# Autodesk Inventor assembly: Batteriepack
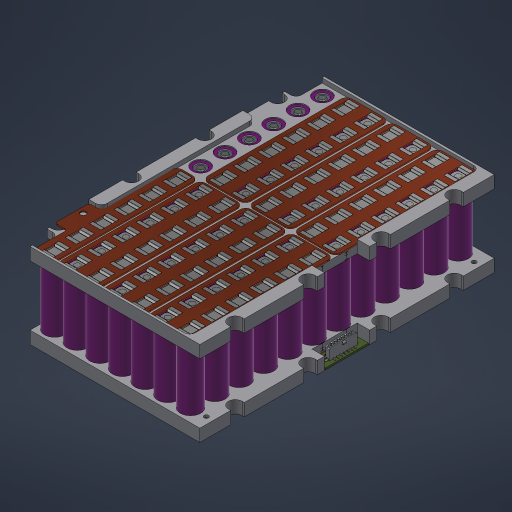
[picture p0: Inventor's stored thumbnail of the model, 512x512]
Saved by Autodesk Inventor 2024.3 (Build 283343010, 343A)
## iProperties
Created: 2025-03-26
Part Number: Batteriepack
Document SubType Name: Assembly
Designer: David Lill
Author: David Lill
## Documents named in this file (8)
- C:\Users\David\Documents\FTAG\E-16\Batterie\Batterie_Konstruktion\E-16 Batterie\Batteriepack.iam
- C:\Users\David\Documents\FTAG\E-16\Batterie\Batterie_Konstruktion\E-16 Batterie\Platte1.ipt
- C:\Users\David\Documents\FTAG\E-16\Batterie\Batterie_Konstruktion\E-16 Batterie\Abstandhalter.ipt
- C:\Users\David\Documents\FTAG\E-16\Batterie\Batterie_Konstruktion\E-16 Batterie\Bat_contacts_v2.iam
- C:\Users\David\Documents\FTAG\E-16\Batterie\Batterie_Konstruktion\E-16 Batterie\18650_assembly.iam
- C:\Users\David\Documents\FTAG\E-16\Batterie\Batterie_Konstruktion\E-16 Batterie\Bat_contacts_v2_long.iam
- C:\Users\David\Documents\FTAG\E-16\Batterie\Batterie_Konstruktion\E-16 Batterie\Platine_unten.ipt
- C:\Users\David\Documents\FTAG\E-16\Batterie\Batterie_Konstruktion\E-16 Batterie\Bat_contacts_v2_contact.iam
## Components (20 placed, 7 different names)
1. Platte1:3 — Einfügen:14, Einfügen:15, Fluchtend:5, Fluchtend:6, Fluchtend:7, Fluchtend:8, Passend:8, Passend:9
2. Platte1:4 — Einfügen:11, Einfügen:12, Einfügen:13, Einfügen:16, Fluchtend:1, Passend:1, Fluchtend:4, Passend:11
3. Abstandhalter:1 — Einfügen:12, Einfügen:14
4. Abstandhalter:2 — Einfügen:11, Einfügen:15
5. 18650_assembly:1 [sub-assembly] — Einfügen:13, Einfügen:16, Passend:6, Passend:7, Passend:10
6. Bat_contacts_v2_long:1 [sub-assembly] — Fluchtend:5, Fluchtend:6, Passend:6, Tangential:1
7. Platine_unten:1 — Passend:8, Passend:9, Tangential:1
8. Bat_contacts_v2_contact:1 [sub-assembly] — Passend:10, Passend:11, Passend:12
9. Bat_contacts_v2:1 [sub-assembly] — Fluchtend:1, Passend:1, Fluchtend:4, Passend:12
10. Bat_contacts_v2:7 [sub-assembly] — Fluchtend:7, Passend:7, Fluchtend:8
11. Bat_contacts_v2:2 [sub-assembly]
12. Bat_contacts_v2:8 [sub-assembly]
13. Bat_contacts_v2:3 [sub-assembly]
14. Bat_contacts_v2:9 [sub-assembly]
15. Bat_contacts_v2:4 [sub-assembly]
16. Bat_contacts_v2:10 [sub-assembly]
17. Bat_contacts_v2:5 [sub-assembly]
18. Bat_contacts_v2:11 [sub-assembly]
19. Bat_contacts_v2:6 [sub-assembly]
20. Bat_contacts_v2:12 [sub-assembly]
## Component patterns: (6 elements, first: Bat_contacts_v2:1 + Bat_contacts_v2:7)
## Relationships (21: Mate 8, Insert 6, Flush 6, Tangent 1)
- Einfügen:11 [Insert]: Platte1:4 ↔ Abstandhalter:2
- Einfügen:12 [Insert]: Platte1:4 ↔ Abstandhalter:1
- Einfügen:13 [Insert]: Platte1:4 ↔ 18650_assembly:1
- Einfügen:14 [Insert]: Platte1:3 ↔ Abstandhalter:1
- Einfügen:15 [Insert]: Platte1:3 ↔ Abstandhalter:2
- Einfügen:16 [Insert]: Platte1:4 ↔ 18650_assembly:1
- Fluchtend:1 [Flush] (2 mm): Platte1:4 ↔ Bat_contacts_v2:1
- Passend:1 [Mate]: Platte1:4 ↔ Bat_contacts_v2:1
- Fluchtend:4 [Flush] (31.5 mm): Platte1:4 ↔ Bat_contacts_v2:1
- Fluchtend:5 [Flush] (11.25 mm): Platte1:3 ↔ Bat_contacts_v2_long:1
- Fluchtend:6 [Flush] (2 mm): Platte1:3 ↔ Bat_contacts_v2_long:1
- Passend:6 [Mate]: 18650_assembly:1 ↔ Bat_contacts_v2_long:1
- Fluchtend:7 [Flush] (11.25 mm): Platte1:3 ↔ Bat_contacts_v2:7
- Passend:7 [Mate]: 18650_assembly:1 ↔ Bat_contacts_v2:7
- Fluchtend:8 [Flush] (2 mm): Platte1:3 ↔ Bat_contacts_v2:7
- Passend:8 [Mate]: Platte1:3 ↔ Platine_unten:1
- Passend:9 [Mate]: Platte1:3 ↔ Platine_unten:1
- Tangential:1: Bat_contacts_v2_long:1 ↔ Platine_unten:1
- Passend:10 [Mate]: 18650_assembly:1 ↔ Bat_contacts_v2_contact:1
- Passend:11 [Mate]: Platte1:4 ↔ Bat_contacts_v2_contact:1
- Passend:12 [Mate] (2 mm): Bat_contacts_v2_contact:1 ↔ Bat_contacts_v2:1
